# Autodesk Inventor assembly: Socket+DIL28
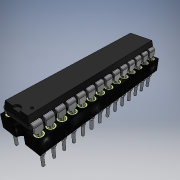
[picture p0: Inventor's stored thumbnail of the model, 180x180]
Saved by Autodesk Inventor 2018 (Build 220112000, 112)
## iProperties
Created: 2020-04-19
Part Number: Socket+DIL28
Material: Všeobecné
Document SubType Name: Assembly
Designer: Jozko Mrkvicka
Author: Jozko Mrkvicka
## Documents named in this file (3)
- F:\Workspace\Projekty\Library\DIL28-Socket+Package.iam
- F:\Workspace\Projekty\Library\DIL28-Package.ipt
- F:\Workspace\Projekty\Library\DIL28-Socket.ipt
## Components (2 placed, 2 different names)
1. DIL28-Package:1 — Vložit:2, Proti sobě:1
2. DIL28-Socket:1 — Vložit:2, Proti sobě:1
## Relationships (2: Insert 1, Mate 1)
- Vložit:2 [Insert]: DIL28-Package:1 ↔ DIL28-Socket:1
- Proti sobě:1 [Mate]: DIL28-Package:1 ↔ DIL28-Socket:1
